# Autodesk Inventor assembly: assembly
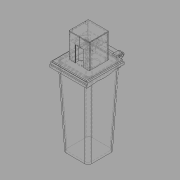
[picture p0: Inventor's stored thumbnail of the model, 180x180]
Saved by Autodesk Inventor 2019 (Build 230136000, 136)
## iProperties
Part Number: assembly
Document SubType Name: Assembly
Designer: Javi
Author: Javi
## Documents named in this file (15)
- D:\MisterBin\assembly.iam
- D:\MisterBin\bin_lid.ipt
- D:\MisterBin\bin_modified.ipt
- D:\MisterBin\lid_holder.ipt
- D:\MisterBin\inner_mechanism.ipt
- D:\MisterBin\security_cover.ipt
- D:\MisterBin\box_front_right.ipt
- D:\MisterBin\box_front_left.ipt
- D:\MisterBin\box_back.ipt
- D:\MisterBin\box_side.ipt
- D:\MisterBin\box_shelf.ipt
- D:\MisterBin\box_top.ipt
- D:\MisterBin\rfid_cover.ipt
- D:\MisterBin\Parallax-Servo_DUMMY.ipt
- D:\MisterBin\Parallax-Servo-Horn.ipt
## Components (16 placed, 14 different names)
1. bin_lid:1 — Insert:1, Insert:2, Insert:4, Insert:5, Rotational:2, Insert:20, Insert:21, Insert:22, Insert:23
2. bin_modified:1 — Rotational:1
3. lid_holder:1 — Insert:1, Insert:2, Rotational:1
4. lid_holder:2 — Insert:4, Insert:5
5. inner_mechanism:1 — Rotational:2, Insert:6, Flush:1
6. security_cover:1 — Insert:6, Flush:1
7. box_front_right:1 — Insert:15, Insert:16, Insert:21
8. box_front_left:1 — Insert:13, Insert:14, Insert:20
9. box_back:1 — Insert:9, Insert:10, Insert:11, Insert:12
10. box_side:1 — Insert:9, Insert:10, Insert:15, Insert:16, Insert:17, Insert:18, Insert:19
11. box_side:2 — Insert:11, Insert:12, Insert:13, Insert:14
12. box_shelf:1 — Insert:17, Insert:18, Insert:25, Insert:26
13. box_top:1 — Insert:19
14. rfid_cover:1 — Insert:22, Insert:23
15. Parallax-Servo_DUMMY:1 — Insert:24, Insert:25, Insert:26
16. Parallax-Servo-Horn:1 — Insert:24
## Relationships (26: Insert 23, RevoluteJoint 2, Flush 1)
- Insert:1: bin_lid:1 ↔ lid_holder:1
- Insert:2: bin_lid:1 ↔ lid_holder:1
- Insert:4: bin_lid:1 ↔ lid_holder:2
- Insert:5: bin_lid:1 ↔ lid_holder:2
- Rotational:1 [RevoluteJoint]: bin_modified:1 ↔ lid_holder:1
- Rotational:2 [RevoluteJoint]: bin_lid:1 ↔ inner_mechanism:1
- Insert:6 (-19.5 mm): inner_mechanism:1 ↔ security_cover:1
- Flush:1: inner_mechanism:1 ↔ security_cover:1
- Insert:9: box_back:1 ↔ box_side:1
- Insert:10: box_back:1 ↔ box_side:1
- Insert:11: box_back:1 ↔ box_side:2
- Insert:12: box_back:1 ↔ box_side:2
- Insert:13: box_front_left:1 ↔ box_side:2
- Insert:14: box_front_left:1 ↔ box_side:2
- Insert:15: box_front_right:1 ↔ box_side:1
- Insert:16: box_front_right:1 ↔ box_side:1
- Insert:17: box_side:1 ↔ box_shelf:1
- Insert:18: box_side:1 ↔ box_shelf:1
- Insert:19: box_side:1 ↔ box_top:1
- Insert:20: bin_lid:1 ↔ box_front_left:1
- Insert:21: bin_lid:1 ↔ box_front_right:1
- Insert:22 (10 mm): bin_lid:1 ↔ rfid_cover:1
- Insert:23 (10 mm): bin_lid:1 ↔ rfid_cover:1
- Insert:24: Parallax-Servo_DUMMY:1 ↔ Parallax-Servo-Horn:1
- Insert:25 (2 mm): box_shelf:1 ↔ Parallax-Servo_DUMMY:1
- Insert:26 (2 mm): box_shelf:1 ↔ Parallax-Servo_DUMMY:1
